# Autodesk Inventor assembly: RT_ARM_A_001
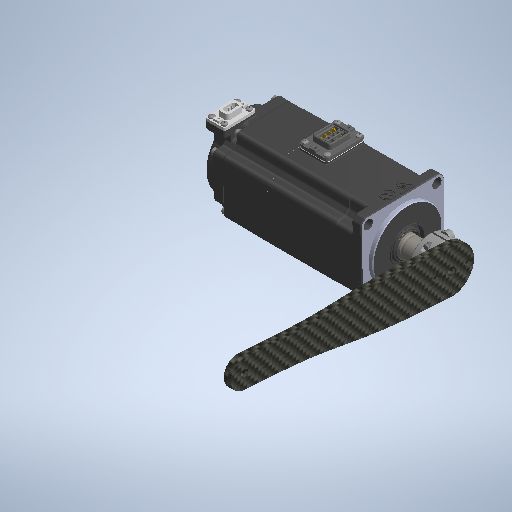
[picture p0: Inventor's stored thumbnail of the model, 512x512]
Saved by Autodesk Inventor 2025.4 (Build 294407000, 407)
## iProperties
Part Number: RT_ARM_A_001
Document SubType Name: Assembly
Designer: louis
Author: louis
## Documents named in this file (6)
- C:\Users\louis\OneDrive\Desktop\R_Trident\02_CAD\04_Subassemblies\RT_ARM_A_001.iam
- C:\Users\louis\OneDrive\Desktop\R_Trident\02_CAD\01_Standard_Parts\623 114 00GA\62311400GA.iam
- C:\Users\louis\OneDrive\Desktop\R_Trident\02_CAD\01_Standard_Parts\CFSTRIP-2-12-2.ipt
- C:\Users\louis\OneDrive\Desktop\R_Trident\02_CAD\03_Parts_Custom\RT_ARM_PR_001.ipt
- C:\Users\louis\OneDrive\Desktop\R_Trident\02_CAD\03_Parts_Custom\RT_ARM_MC_002.ipt
- C:\Users\louis\OneDrive\Desktop\R_Trident\02_CAD\01_Standard_Parts\A6M60-400H2B1-M17\A6M60-400H2B1-M17.iam
## Components (6 placed, 5 different names)
1. 62311400GA:1 [sub-assembly] — Mate:1, Flush:3, Mate:4, Mate:5, Mate:6, Mate:7
2. CFSTRIP-2-12-2:1 — Mate:3
3. CFSTRIP-2-12-2:2 — Mate:2
4. RT_ARM_PR_001:1 — Mate:2, Mate:3, Mate:4
5. RT_ARM_MC_002:1 — Mate:5, Mate:6, Mate:8
6. A6M60-400H2B1-M17:1 [sub-assembly] — Mate:7, Mate:8
## Relationships (9: Mate 8, Flush 1)
- Mate:1: 62311400GA:1
- Flush:3: 62311400GA:1
- Mate:2: CFSTRIP-2-12-2:2 ↔ RT_ARM_PR_001:1
- Mate:3: CFSTRIP-2-12-2:1 ↔ RT_ARM_PR_001:1
- Mate:4: 62311400GA:1 ↔ RT_ARM_PR_001:1
- Mate:5: 62311400GA:1 ↔ RT_ARM_MC_002:1
- Mate:6: 62311400GA:1 ↔ RT_ARM_MC_002:1
- Mate:7: 62311400GA:1 ↔ A6M60-400H2B1-M17:1
- Mate:8: RT_ARM_MC_002:1 ↔ A6M60-400H2B1-M17:1
